# Autodesk Inventor assembly: Frame
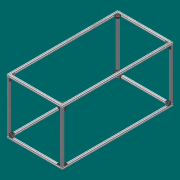
[picture p0: Inventor's stored thumbnail of the model, 180x180]
Saved by Autodesk Inventor 2016 (Build 200138000, 138)
## iProperties
Created: 2015-06-02
Part Number: Frame
Document SubType Name: Assembly
Designer: Sawaiz Syed
Author: Sawaiz Syed
## Documents named in this file (3)
- C:\Users\Sawaiz\Documents\data\projects\cncBlackBox\frame\Frame.iam
- C:\Users\Sawaiz\Documents\data\projects\cncBlackBox\frame\frameHorizontal.iam
- C:\Users\Sawaiz\Documents\data\projects\cncBlackBox\frame\verticalStrut.iam
## Components (6 placed, 2 different names)
1. frameHorizontal:1 [sub-assembly] — Mate:1, Flush:1, Flush:2, Flush:3, Flush:4, Flush:7, Flush:8, Flush:9, Flush:10
2. frameHorizontal:2 [sub-assembly] — Flush:5, Flush:6, Mate:2
3. verticalStrut:1 [sub-assembly] — Flush:3, Flush:4, Flush:5, Flush:6, Flush:12, Flush:13
4. verticalStrut:2 [sub-assembly] — Flush:7, Flush:8, Flush:11, Flush:12
5. verticalStrut:3 [sub-assembly] — Flush:9, Flush:10, Flush:11
6. verticalStrut:4 [sub-assembly] — Mate:1, Flush:1, Flush:2, Mate:2, Flush:13
## Relationships (15: Flush 13, Mate 2)
- Mate:1: frameHorizontal:1 ↔ verticalStrut:4
- Flush:1: frameHorizontal:1 ↔ verticalStrut:4
- Flush:2: frameHorizontal:1 ↔ verticalStrut:4
- Flush:3: frameHorizontal:1 ↔ verticalStrut:1
- Flush:4: frameHorizontal:1 ↔ verticalStrut:1
- Flush:5: frameHorizontal:2 ↔ verticalStrut:1
- Flush:6: frameHorizontal:2 ↔ verticalStrut:1
- Flush:7: frameHorizontal:1 ↔ verticalStrut:2
- Flush:8: frameHorizontal:1 ↔ verticalStrut:2
- Flush:9: frameHorizontal:1 ↔ verticalStrut:3
- Flush:10: frameHorizontal:1 ↔ verticalStrut:3
- Mate:2: frameHorizontal:2 ↔ verticalStrut:4
- Flush:11: verticalStrut:2 ↔ verticalStrut:3
- Flush:12: verticalStrut:1 ↔ verticalStrut:2
- Flush:13: verticalStrut:1 ↔ verticalStrut:4
